# Autodesk Inventor assembly: full Assembly new
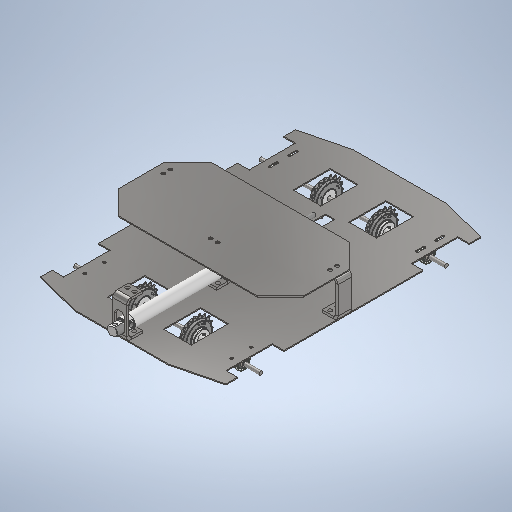
[picture p0: Inventor's stored thumbnail of the model, 512x512]
Saved by Autodesk Inventor 2026.1 (Build 301233020, 233B)
## iProperties
Created: 2026-01-25
Part Number: full Assembly new
Document SubType Name: Assembly
Designer: user
Author: user
## Documents named in this file (8)
- D:\asu\machine element design\project\design - Copy\full Assembly new.iam
- D:\asu\machine element design\project\design - Copy\chassis.ipt
- D:\asu\machine element design\project\design - Copy\piston bracket.ipt
- D:\asu\machine element design\project\design - Copy\up bracket.ipt
- D:\asu\machine element design\project\design - Copy\pillow-block-bearing-p08-1.snapshot.17\Pillow Block P08\Pillow Block P08\Pillow Block P08.ipt
- D:\asu\machine element design\project\design - Copy\Assembly shaft 1 sprocect.iam
- D:\asu\machine element design\project\design - Copy\piston\piston .iam
- D:\asu\machine element design\project\design - Copy\chassis up .ipt
## Components (13 placed, 7 different names)
1. chassis:1 — Mate:1, Mate:2, Mate:3, Mate:4, Mate:5, Mate:6, Mate:7, Mate:8, Mate:9, Mate:10, Mate:11, Mate:12, Mate:13, Mate:14, Mate:15, Mate:16, Mate:17, Mate:18, Mate:19, Mate:20, Mate:21, Mate:22, Mate:23, Mate:24
2. piston bracket:1 — Mate:8, Mate:11, Mate:12, Mate:29
3. up bracket:1 — Mate:4, Mate:5, Mate:6, Mate:32, Mate:33
4. piston bracket:2 — Mate:7, Mate:9, Mate:10, Mate:30
5. up bracket:2 — Mate:1, Mate:2, Mate:3, Mate:31
6. Pillow Block P08:1 — Mate:19, Mate:20, Mate:21
7. Pillow Block P08:2 — Mate:13, Mate:14, Mate:15
8. Pillow Block P08:3 — Mate:16, Mate:17, Mate:18, Mate:25, Mate:26
9. Pillow Block P08:4 — Mate:22, Mate:23, Mate:24, Mate:27, Mate:28
10. Assembly shaft 1 sprocect:1 [sub-assembly] — Mate:25, Mate:26
11. Assembly shaft 1 sprocect:2 [sub-assembly] — Mate:27, Mate:28
12. piston :1 [sub-assembly] — Mate:29, Mate:30
13. chassis up :1 — Mate:31, Mate:32, Mate:33
## Relationships (33: Mate 33)
- Mate:1: chassis:1 ↔ up bracket:2
- Mate:2: chassis:1 ↔ up bracket:2
- Mate:3: chassis:1 ↔ up bracket:2
- Mate:4: chassis:1 ↔ up bracket:1
- Mate:5: chassis:1 ↔ up bracket:1
- Mate:6: chassis:1 ↔ up bracket:1
- Mate:7: chassis:1 ↔ piston bracket:2
- Mate:8: chassis:1 ↔ piston bracket:1
- Mate:9: chassis:1 ↔ piston bracket:2
- Mate:10: chassis:1 ↔ piston bracket:2
- Mate:11: chassis:1 ↔ piston bracket:1
- Mate:12: chassis:1 ↔ piston bracket:1
- Mate:13: chassis:1 ↔ Pillow Block P08:2
- Mate:14: chassis:1 ↔ Pillow Block P08:2
- Mate:15: chassis:1 ↔ Pillow Block P08:2
- Mate:16: chassis:1 ↔ Pillow Block P08:3
- Mate:17: chassis:1 ↔ Pillow Block P08:3
- Mate:18: chassis:1 ↔ Pillow Block P08:3
- Mate:19: chassis:1 ↔ Pillow Block P08:1
- Mate:20: chassis:1 ↔ Pillow Block P08:1
- Mate:21: chassis:1 ↔ Pillow Block P08:1
- Mate:22: chassis:1 ↔ Pillow Block P08:4
- Mate:23: chassis:1 ↔ Pillow Block P08:4
- Mate:24: chassis:1 ↔ Pillow Block P08:4
- Mate:25: Pillow Block P08:3 ↔ Assembly shaft 1 sprocect:1
- Mate:26 (72 mm): Pillow Block P08:3 ↔ Assembly shaft 1 sprocect:1
- Mate:27: Pillow Block P08:4 ↔ Assembly shaft 1 sprocect:2
- Mate:28 (72 mm): Pillow Block P08:4 ↔ Assembly shaft 1 sprocect:2
- Mate:29: piston bracket:1 ↔ piston :1
- Mate:30: piston bracket:2 ↔ piston :1
- Mate:31: up bracket:2 ↔ chassis up :1
- Mate:32: up bracket:1 ↔ chassis up :1
- Mate:33: up bracket:1 ↔ chassis up :1
